# Autodesk Inventor assembly: Bateria+Podkladka
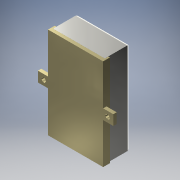
[picture p0: Inventor's stored thumbnail of the model, 180x180]
Saved by Autodesk Inventor 2017 (Build 210142000, 142)
## iProperties
Created: 2016-11-21
Part Number: Bateria+Podkladka
Document SubType Name: Assembly
Designer: Shichi
Author: Shichi
## Documents named in this file (3)
- C:\Users\Shichi\Desktop\TooStronk\Bateria\Bateria+Podkladka.iam
- C:\Users\Shichi\Desktop\TooStronk\Bateria\Bateria_Podkladka.ipt
- C:\Users\Shichi\Desktop\TooStronk\Bateria\Bateria.ipt
## Components (2 placed, 2 different names)
1. Bateria_Podkladka:1 — Mate:1, Mate:2
2. Bateria:1 — Mate:1, Mate:2
## Relationships (2: Mate 2)
- Mate:1: Bateria_Podkladka:1 ↔ Bateria:1
- Mate:2: Bateria_Podkladka:1 ↔ Bateria:1
